# Autodesk Inventor assembly: top_roller_bearing
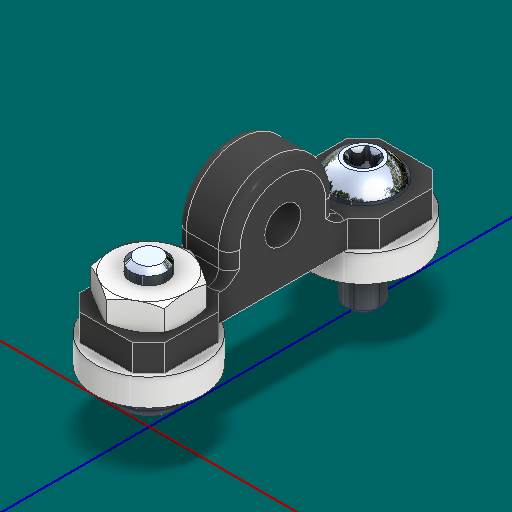
[picture p0: Inventor's stored thumbnail of the model, 512x512]
Saved by Autodesk Inventor 2025 (Build 290162000, 162)
## iProperties
Created: 2024-08-18
Part Number: top_roller_bearing
Document SubType Name: Assembly
Designer: averey
Author: averey
## Documents named in this file (8)
- C:\Users\avere\vex_robotics_high_stakes\hardware\cad\ATLAS\intake\first_stage\top_roller_bearing.iam
- C:\Users\avere\vex_robotics_high_stakes\hardware\cad\VEX-CAD-Inventor\Motion\Shaft LS\LS Pillow Bearing Block.ipt
- C:\Users\avere\vex_robotics_high_stakes\hardware\cad\VEX-CAD-Inventor\Motion\Spacers\Spacer Nylon .500 OD\NSpacer White .500 OD x .125.ipt
- C:\Users\avere\vex_robotics_high_stakes\hardware\cad\VEX-CAD-Inventor\Motion\Spacers\Spacer Nylon .500 OD.ipt
- C:\Users\avere\vex_robotics_high_stakes\hardware\cad\VEX-CAD-Inventor\Structure\Hardware\Screw Shoulder Robosource\SScrew Shoulder Smooth .500 x .18.ipt
- C:\Users\avere\vex_robotics_high_stakes\hardware\cad\VEX-CAD-Inventor\Structure\Hardware\Screw Shoulder Robosource.ipt
- C:\Users\avere\vex_robotics_high_stakes\hardware\cad\VEX-CAD-Inventor\Structure\Hardware\Nut Nylon\Nut Nylon - White.ipt
- C:\Users\avere\vex_robotics_high_stakes\hardware\cad\VEX-CAD-Inventor\Structure\Hardware\Nut Nylon.ipt
## Components (6 placed, 4 different names)
1. LS Pillow Bearing Block:1 — Insert:6
2. NSpacer White .500 OD x .125:1
3. NSpacer White .500 OD x .125:2 — Mate:1, Insert:5
4. SScrew Shoulder Smooth .500 x .18:1
5. SScrew Shoulder Smooth .500 x .18:2 — Insert:5
6. Nut Nylon - White:1 — Insert:6
## Relationships (6: Insert 5, Mate 1)
- [Insert]: LS Pillow Bearing Block:1 ↔ SScrew Shoulder Smooth .500 x .18:1
- [Insert]: LS Pillow Bearing Block:1 ↔ NSpacer White .500 OD x .125:2
- [Insert]: LS Pillow Bearing Block:1 ↔ NSpacer White .500 OD x .125:1
- Mate:1: NSpacer White .500 OD x .125:2
- Insert:5 (1.5875 mm): NSpacer White .500 OD x .125:2 ↔ SScrew Shoulder Smooth .500 x .18:2
- Insert:6: LS Pillow Bearing Block:1 ↔ Nut Nylon - White:1
